# Autodesk Inventor assembly: Sideassembly_MIR
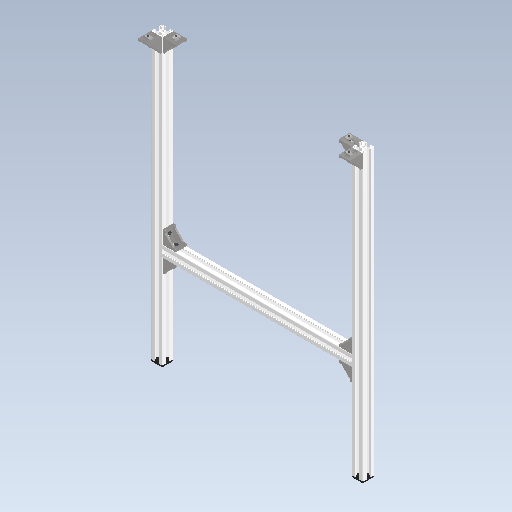
[picture p0: Inventor's stored thumbnail of the model, 512x512]
Saved by Autodesk Inventor 2020.2 (Build 242310000, 310)
## iProperties
Created: 2020-07-25
Part Number: Sideassembly_MIR
Document SubType Name: Assembly
Designer: JK
Author: JK
## Documents named in this file (3)
- C:\Users\JK\Documents\Inventor\Mesa\Sideassembly_MIR.iam
- C:\Users\JK\Documents\Inventor\Mesa\Legassembly_MIR.iam
- C:\Users\JK\Documents\Inventor\Mesa\Legstretcher_MIR.iam
## Components (3 placed, 2 different names)
1. Legassembly_MIR:1 [sub-assembly] — Flush:3, Flush:1, Mate:1
2. Legassembly_MIR:2 [sub-assembly] — Flush:3, Flush:4, Flush:2, Mate:2
3. Legstretcher_MIR:1 [sub-assembly] — Flush:4, Flush:2, Mate:2, Flush:1, Mate:1
## Relationships (6: Flush 4, Mate 2)
- Flush:3: Legassembly_MIR:1 ↔ Legassembly_MIR:2
- Flush:4 (250 mm): Legassembly_MIR:2 ↔ Legstretcher_MIR:1
- Flush:2 (0.5 mm): Legassembly_MIR:2 ↔ Legstretcher_MIR:1
- Mate:2: Legassembly_MIR:2 ↔ Legstretcher_MIR:1
- Flush:1 (0.5 mm): Legassembly_MIR:1 ↔ Legstretcher_MIR:1
- Mate:1: Legassembly_MIR:1 ↔ Legstretcher_MIR:1
